# Autodesk Inventor assembly: steering_kingpin_left_assy
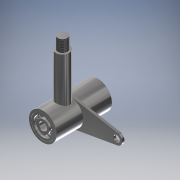
[picture p0: Inventor's stored thumbnail of the model, 180x180]
Saved by Autodesk Inventor 2019 (Build 230136000, 136)
## iProperties
Created: 2019-04-24
Part Number: steering_kingpin_left_assy
Document SubType Name: Assembly
Designer: callum.snowden
Author: callum.snowden
## Documents named in this file (4)
- C:\Users\callum.snowden\Documents\GitHub\clasohlsonkart\mechanical\frame\steering_kingpin_left_assy.iam
- C:\Users\callum.snowden\Documents\GitHub\clasohlsonkart\mechanical\frame\steering_kingpin_left.ipt
- C:\Users\callum.snowden\Documents\Inventor\Content Center Files\R2019\en-US\SKF 2Z - with two shields\SKF 2Z6200-2Z.ipt
- C:\Users\callum.snowden\Documents\GitHub\clasohlsonkart\mechanical\frame\steering_kingpin_bearing_spacer.ipt
## Components (4 placed, 3 different names)
1. steering_kingpin_left:1 — Rigid:1, Rigid:3
2. SKF 2Z- with two shields SKF 2Z6200-2Z:1 — Rigid:3
3. SKF 2Z- with two shields SKF 2Z6200-2Z:2 — Rigid:1, Rigid:2
4. steering_kingpin_bearing_spacer:1 — Rigid:2
## Relationships (3: WeldJoint 3)
- Rigid:1 [WeldJoint]: steering_kingpin_left:1 ↔ SKF 2Z- with two shields SKF 2Z6200-2Z:2
- Rigid:2 [WeldJoint]: SKF 2Z- with two shields SKF 2Z6200-2Z:2 ↔ steering_kingpin_bearing_spacer:1
- Rigid:3 [WeldJoint]: steering_kingpin_left:1 ↔ SKF 2Z- with two shields SKF 2Z6200-2Z:1
